# Autodesk Inventor assembly: SPM
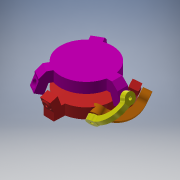
[picture p0: Inventor's stored thumbnail of the model, 180x180]
Saved by Autodesk Inventor 2019 (Build 230136000, 136)
## iProperties
Created: 2022-07-05
Part Number: SPM
Document SubType Name: Assembly
Designer: zreik
Author: zreik
## Documents named in this file (6)
- D:\Documents\HIAST\4th year\4th Year Project\Design\SPM.iam
- D:\Documents\HIAST\4th year\4th Year Project\Design\Platform.ipt
- D:\Documents\HIAST\4th year\4th Year Project\Design\Link.ipt
- D:\Documents\HIAST\4th year\4th Year Project\Design\Link2.ipt
- D:\Documents\HIAST\4th year\4th Year Project\Design\BottomPlatform.ipt
- D:\Documents\HIAST\4th year\4th Year Project\Design\TopPlatform.ipt
## Components (9 placed, 5 different names)
1. Platform:2 — Mate:15, Mate:16, Mate:17, Mate:18, Mate:32
2. Link:1 — Mate:19, Mate:20
3. Link:2 — Mate:21, Mate:22, Mate:30, Mate:31
4. Link:3 — Mate:13, Mate:14
5. Link2:1 — Mate:13, Mate:14, Mate:15, Mate:16
6. Link2:2 — Mate:17, Mate:18, Mate:19, Mate:20
7. Link2:3 — Mate:21, Mate:22, Mate:34, Mate:35
8. BottomPlatform:1 — Flush:26, Mate:26, Mate:27, Mate:30, Mate:31, Mate:32, Mate:36
9. TopPlatform:1 — Mate:34, Mate:35, Mate:36
## Relationships (19: Mate 18, Flush 1)
- Mate:13: Link:3 ↔ Link2:1
- Mate:14: Link:3 ↔ Link2:1
- Mate:15: Platform:2 ↔ Link2:1
- Mate:16: Platform:2 ↔ Link2:1
- Mate:17: Platform:2 ↔ Link2:2
- Mate:18: Platform:2 ↔ Link2:2
- Mate:19: Link:1 ↔ Link2:2
- Mate:20: Link:1 ↔ Link2:2
- Mate:21: Link:2 ↔ Link2:3
- Mate:22: Link:2 ↔ Link2:3
- Flush:26: BottomPlatform:1
- Mate:26: BottomPlatform:1
- Mate:27: BottomPlatform:1
- Mate:30: Link:2 ↔ BottomPlatform:1
- Mate:31: Link:2 ↔ BottomPlatform:1
- Mate:32: Platform:2 ↔ BottomPlatform:1
- Mate:34: Link2:3 ↔ TopPlatform:1
- Mate:35: Link2:3 ↔ TopPlatform:1
- Mate:36: BottomPlatform:1 ↔ TopPlatform:1
